# Autodesk Inventor assembly: ASY GBK bottom 0023
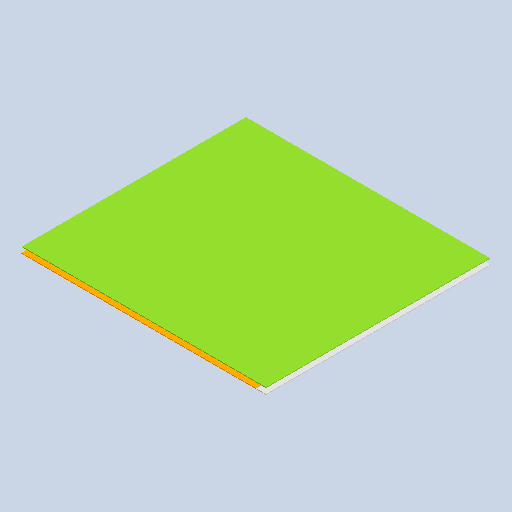
[picture p0: Inventor's stored thumbnail of the model, 512x512]
Saved by Autodesk Inventor 2026 (Build 300175000, 175)
## iProperties
Created: 2026-07-15
Part Number: ASY GBK bottom 0023
Document SubType Name: Assembly
Designer: user
Author: user
## Documents named in this file (4)
- C:\Users\user\Documents\Inventor\GBK-Gubkinskiy\ASY GBK bottom 0023.iam
- C:\Users\user\Documents\Inventor\GBK-Gubkinskiy\Пол\GBK bottom 0124.ipt
- C:\Users\user\Documents\Inventor\GBK-Gubkinskiy\Пол\GBK bottom 0133.ipt
- C:\Users\user\Documents\Inventor\GBK-Gubkinskiy\Пол\GBK bottom 0134.ipt
## Components (3 placed, 3 different names)
1. GBK bottom 0124:1
2. GBK 0214  bottom:1
3. GBK bottom 0134:1
## Relationships (4: Mate 3, WeldJoint 1)
- [Mate]: GBK bottom 0124:1 ↔ GBK 0214  bottom:1
- [Mate] (-30 mm): GBK bottom 0124:1 ↔ GBK bottom 0134:1
- [WeldJoint]: GBK 0214  bottom:1 ↔ GBK bottom 0134:1
- [Mate] (-30 mm): GBK bottom 0124:1 ↔ GBK 0214  bottom:1
